# Autodesk Inventor assembly: R6_assembly
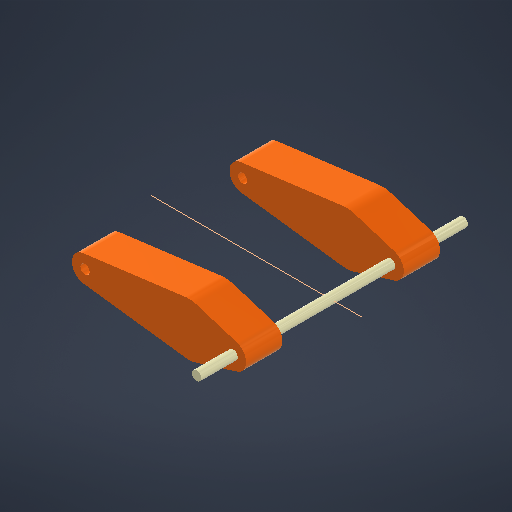
[picture p0: Inventor's stored thumbnail of the model, 512x512]
Saved by Autodesk Inventor 2025.3 (Build 293356030, 356C)
## iProperties
Created: 2025-09-01
Part Number: R6_assembly
Document SubType Name: Assembly
Designer: 陳泓任
Author: 陳泓任
## Documents named in this file (3)
- C:\Users\Ou918\Downloads\AI-optimization\reference\model\R5_assembly.iam
- C:\Users\Ou918\Downloads\AI-optimization\reference\model\Type 1A R5主滑台連接桿.ipt
- C:\Users\Ou918\Downloads\AI-optimization\reference\model\Type 1A 連接軸 1.ipt
## Components (2 placed, 2 different names)
1. Type 1A R5主滑台連接桿:1 — 插入:1, 角度:1
2. Type 1A 連接軸 1:1 — 插入:1, 角度:1
## Relationships (2: Insert 1, Angle 1)
- 插入:1 [Insert] (-103 mm): Type 1A R5主滑台連接桿:1 ↔ Type 1A 連接軸 1:1
- 角度:1 [Angle] (0 deg): Type 1A R5主滑台連接桿:1 ↔ Type 1A 連接軸 1:1
